# Autodesk Inventor assembly: Right shoulder
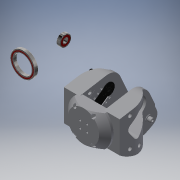
[picture p0: Inventor's stored thumbnail of the model, 180x180]
Saved by Autodesk Inventor 2017 (Build 210142000, 142)
## iProperties
Created: 2016-08-11
Part Number: Right shoulder
Document SubType Name: Assembly
Designer: Ali
Author: Ali
## Documents named in this file (8)
- C:\Users\Alistair\Dropbox\Work\Project\Inventor\Right shoulder.iam
- C:\Users\Alistair\Dropbox\Work\Project\Inventor\Arm - right shoulder v3.ipt
- C:\Users\Alistair\Dropbox\Work\Project\Inventor\ax12_box.ipt
- C:\Users\Alistair\Dropbox\Work\Project\Inventor\ax12_wheel.ipt
- C:\Users\Alistair\Dropbox\Work\Project\Inventor\Arm - left shoulder v3.ipt
- C:\Users\Alistair\Dropbox\Work\Project\Inventor\Arm - base v3.ipt
- C:\Users\Alistair\Dropbox\Work\Project\Inventor\Parts\68072RS.iam
- C:\Users\Alistair\Dropbox\Work\Project\Inventor\Parts\6082RS.iam
## Components (7 placed, 7 different names)
1. Arm - right shoulder v3:1 — Rigid:1, Rigid:2
2. ax12_box:1 — Rigid:1, Rotational:1
3. ax12_wheel:1 — Rotational:1
4. Arm - left shoulder v3:1 — Rigid:3
5. Arm - base v3:1 — Rigid:2, Rigid:3
6. 68072RS:1 [sub-assembly]
7. 6082RS:1 [sub-assembly]
## Relationships (4: WeldJoint 3, RevoluteJoint 1)
- Rigid:1 [WeldJoint]: Arm - right shoulder v3:1 ↔ ax12_box:1
- Rotational:1 [RevoluteJoint]: ax12_box:1 ↔ ax12_wheel:1
- Rigid:2 [WeldJoint]: Arm - right shoulder v3:1 ↔ Arm - base v3:1
- Rigid:3 [WeldJoint]: Arm - left shoulder v3:1 ↔ Arm - base v3:1
